# Autodesk Inventor assembly: FullAssembly
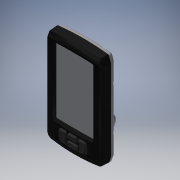
[picture p0: Inventor's stored thumbnail of the model, 180x180]
Saved by Autodesk Inventor 2018 (Build 220112000, 112)
## iProperties
Created: 2019-05-29
Part Number: FullAssembly
Document SubType Name: Assembly
Designer: Ash
Author: Ash
## Documents named in this file (8)
- C:\Autodesk\Skills 2019 Nationals\Competition\GivenFiles\Day 2 AM\Day 2 AM\FullAssembly.iam
- C:\Autodesk\Skills 2019 Nationals\Competition\AMDay2\96710A373_STAINLESS STEEL PAN HEAD TORX SCREWS.ipt
- C:\Autodesk\Skills 2019 Nationals\Competition\AMDay2\410141-1.ipt
- C:\Autodesk\Skills 2019 Nationals\Competition\AMDay2\410142.ipt
- C:\Autodesk\Skills 2019 Nationals\Competition\AMDay2\410153-1_ASM.iam
- C:\Autodesk\Skills 2019 Nationals\Competition\AMDay2\410154-1_ASSY_DISP_PMAX4.ipt
- C:\Autodesk\Skills 2019 Nationals\Competition\AMDay2\472147-1.ipt
- C:\Autodesk\Skills 2019 Nationals\Competition\AMDay2\GASKET.ipt
## Components (14 placed, 7 different names)
1. 96710A373_STAINLESS STEEL PAN HEAD TORX SCREWS:1 — Mate:11, Mate:12
2. 410141-1:1 — Mate:4, Mate:5, Mate:6, Mate:7, Mate:8, Mate:9, Mate:10
3. 410142:1 — Mate:4
4. 410153-1_ASM:1 [sub-assembly] — Mate:1, Mate:2, Mate:3, Mate:9, Mate:10, Mate:11, Mate:12, Mate:13, Mate:14, Mate:15, Mate:16, Mate:17, Mate:18, Mate:19, Mate:20, Mate:21, Mate:22, Mate:23, Mate:24, Mate:25, Mate:26
5. 410154-1_ASSY_DISP_PMAX4:1 — Mate:7
6. 472147-1:1 — Mate:5, Mate:6
7. GASKET:1 — Mate:1, Mate:2, Mate:3, Mate:8
8. 96710A373_STAINLESS STEEL PAN HEAD TORX SCREWS:2 — Mate:15, Mate:16
9. 96710A373_STAINLESS STEEL PAN HEAD TORX SCREWS:3 — Mate:13, Mate:14
10. 96710A373_STAINLESS STEEL PAN HEAD TORX SCREWS:4 — Mate:21, Mate:22
11. 96710A373_STAINLESS STEEL PAN HEAD TORX SCREWS:5 — Mate:18, Mate:25
12. 96710A373_STAINLESS STEEL PAN HEAD TORX SCREWS:6 — Mate:17, Mate:26
13. 96710A373_STAINLESS STEEL PAN HEAD TORX SCREWS:7 — Mate:19, Mate:24
14. 96710A373_STAINLESS STEEL PAN HEAD TORX SCREWS:8 — Mate:20, Mate:23
## Relationships (26: Mate 26)
- Mate:1: 410153-1_ASM:1 ↔ GASKET:1
- Mate:2: 410153-1_ASM:1 ↔ GASKET:1
- Mate:3: 410153-1_ASM:1 ↔ GASKET:1
- Mate:4: 410141-1:1 ↔ 410142:1
- Mate:5: 410141-1:1 ↔ 472147-1:1
- Mate:6: 410141-1:1 ↔ 472147-1:1
- Mate:7: 410141-1:1 ↔ 410154-1_ASSY_DISP_PMAX4:1
- Mate:8: 410141-1:1 ↔ GASKET:1
- Mate:9: 410141-1:1 ↔ 410153-1_ASM:1
- Mate:10: 410141-1:1 ↔ 410153-1_ASM:1
- Mate:11: 96710A373_STAINLESS STEEL PAN HEAD TORX SCREWS:1 ↔ 410153-1_ASM:1
- Mate:12: 96710A373_STAINLESS STEEL PAN HEAD TORX SCREWS:1 ↔ 410153-1_ASM:1
- Mate:13: 410153-1_ASM:1 ↔ 96710A373_STAINLESS STEEL PAN HEAD TORX SCREWS:3
- Mate:14: 410153-1_ASM:1 ↔ 96710A373_STAINLESS STEEL PAN HEAD TORX SCREWS:3
- Mate:15: 410153-1_ASM:1 ↔ 96710A373_STAINLESS STEEL PAN HEAD TORX SCREWS:2
- Mate:16: 410153-1_ASM:1 ↔ 96710A373_STAINLESS STEEL PAN HEAD TORX SCREWS:2
- Mate:17: 410153-1_ASM:1 ↔ 96710A373_STAINLESS STEEL PAN HEAD TORX SCREWS:6
- Mate:18: 410153-1_ASM:1 ↔ 96710A373_STAINLESS STEEL PAN HEAD TORX SCREWS:5
- Mate:19: 410153-1_ASM:1 ↔ 96710A373_STAINLESS STEEL PAN HEAD TORX SCREWS:7
- Mate:20: 410153-1_ASM:1 ↔ 96710A373_STAINLESS STEEL PAN HEAD TORX SCREWS:8
- Mate:21: 410153-1_ASM:1 ↔ 96710A373_STAINLESS STEEL PAN HEAD TORX SCREWS:4
- Mate:22: 410153-1_ASM:1 ↔ 96710A373_STAINLESS STEEL PAN HEAD TORX SCREWS:4
- Mate:23: 410153-1_ASM:1 ↔ 96710A373_STAINLESS STEEL PAN HEAD TORX SCREWS:8
- Mate:24: 410153-1_ASM:1 ↔ 96710A373_STAINLESS STEEL PAN HEAD TORX SCREWS:7
- Mate:25: 410153-1_ASM:1 ↔ 96710A373_STAINLESS STEEL PAN HEAD TORX SCREWS:5
- Mate:26: 410153-1_ASM:1 ↔ 96710A373_STAINLESS STEEL PAN HEAD TORX SCREWS:6
